# Autodesk Inventor assembly: ENGRANAJES GUSANO BRAZO COPIA SEGURIDAD 30.7
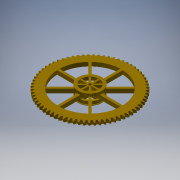
[picture p0: Inventor's stored thumbnail of the model, 180x180]
Saved by Autodesk Inventor 2016 (Build 200138000, 138)
## iProperties
Created: 2016-07-30
Part Number: ENGRANAJES GUSANO BRAZO COPIA SEGURIDAD 30.7
Document SubType Name: Assembly
Designer: Admin
Author: Admin
## Documents named in this file (6)
- C:\Users\Admin\Dropbox\diseños autodesk dimer\ENGRANAJES GUSANO BRAZO COPIA SEGURIDAD 30.7.iam
- C:\Users\Admin\Dropbox\diseños autodesk dimer\soporte worm.ipt
- C:\Users\Admin\Dropbox\diseños autodesk dimer\worm gear\Design Accelerator\Worm Gears2.iam
- C:\Users\Admin\Dropbox\diseños autodesk dimer\worm gear\Design Accelerator\Spur Gears2.iam
- C:\Users\Admin\Dropbox\diseños autodesk dimer\worm gear\Design Accelerator\Spur Gears1.iam
- C:\Users\Admin\Dropbox\diseños autodesk dimer\ENGRANAJES GUSANO BRAZO COPIA SEGURIDAD 30.7\Design Accelerator\Worm Gears4.iam
## Components (7 placed, 3 different names)
1. Worm Gears:1 [sub-assembly] — Tangent:1
2. Spur Gears:1 [sub-assembly] — Flush:2, Mate:3
3. Spur Gears:2 [sub-assembly] — Flush:2, Mate:3, Mate:4, Mate:5
4. soporte worm:1 — Tangent:1
5. soporte worm:2
6. Worm Gears:2 [sub-assembly] — Mate:4, Mate:5, Mate:6, Mate:7
7. Spur Gears:3 [sub-assembly] — Mate:6, Mate:7
## Relationships (7: Mate 5, Flush 1, Tangent 1)
- Flush:2: Spur Gears:1 ↔ Spur Gears:2
- Mate:3 (400 mm): Spur Gears:1 ↔ Spur Gears:2
- Tangent:1: Worm Gears:1 ↔ soporte worm:1
- Mate:4: Spur Gears:2 ↔ Worm Gears:2
- Mate:5: Spur Gears:2 ↔ Worm Gears:2
- Mate:6: Worm Gears:2 ↔ Spur Gears:3
- Mate:7: Worm Gears:2 ↔ Spur Gears:3
